# Autodesk Inventor assembly: Stufen Zusammenbau
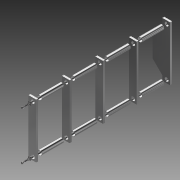
[picture p0: Inventor's stored thumbnail of the model, 180x180]
Saved by Autodesk Inventor 2019 (Build 230136000, 136)
## iProperties
Created: 2020-05-13
Part Number: Stufen Zusammenbau
Material: Generisch
Document SubType Name: Assembly
Designer: seele
Author: seele
## Documents named in this file (7)
- F:\Desktop\Neuer Ordner\Zubehör\Badeleiter\Stufen Zusammenbau.iam
- F:\Desktop\Neuer Ordner\Zubehör\Badeleiter\Tritt.ipt
- F:\Desktop\Neuer Ordner\Zubehör\Badeleiter\Tritt oben.ipt
- F:\Desktop\Neuer Ordner\Zubehör\Badeleiter\Stufenrohr.ipt
- C:\Users\seele\Documents\Inventor\Content Center Files\R2019\de-DE\DIN 931-1\DIN 931-1 - M12 x 50.ipt
- C:\Users\seele\Documents\Inventor\Content Center Files\R2019\de-DE\DIN 128\DIN 128 - A12.ipt
- C:\Users\seele\Documents\Inventor\Content Center Files\R2019\de-DE\DIN 9021\DIN 9021 - 13.ipt
## Components (19 placed, 6 different names)
1. Tritt:1 — Fluchtend:1, Fluchtend:6, Passend:1, Passend:9, Passend:30, Passend:31, Passend:32
2. Tritt:2 — Fluchtend:1, Fluchtend:2, Fluchtend:5, Fluchtend:6, Passend:2, Passend:8, Passend:10, Passend:11
3. Tritt:3 — Fluchtend:2, Fluchtend:3, Fluchtend:4, Fluchtend:5, Passend:3, Passend:7, Passend:12, Passend:13
4. Tritt:4 — Fluchtend:3, Fluchtend:4, Fluchtend:7, Fluchtend:8, Passend:6, Passend:14, Passend:15
5. Tritt oben:1 — Fluchtend:7, Fluchtend:8, Passend:4, Passend:5, Passend:16
6. Stufenrohr:1 — Passend:4, Passend:15, Passend:16, Fluchtend:9
7. Stufenrohr:2 — Passend:5, Fluchtend:9
8. Stufenrohr:3 — Passend:6, Fluchtend:10
9. Stufenrohr:4 — Passend:3, Passend:13, Passend:14, Fluchtend:10
10. Stufenrohr:5 — Passend:2, Passend:11, Passend:12, Fluchtend:11
11. Stufenrohr:6 — Passend:7, Fluchtend:11
12. Stufenrohr:7 — Passend:8, Fluchtend:12
13. Stufenrohr:8 — Passend:1, Passend:9, Passend:10, Fluchtend:12
14. DIN 931-1 - ersetzt durch DIN EN 24014 M12 x 50:3 — Passend:25, Passend:30, Fluchtend:13
15. DIN 128 A12:3
16. DIN 9021 13:1 — Passend:25, Passend:32
17. DIN 931-1 - ersetzt durch DIN EN 24014 M12 x 50:4 — Passend:31, Fluchtend:13
18. DIN 128 A12:4
19. DIN 9021 13:2
## Relationships (40: Mate 27, Flush 13)
- Fluchtend:1 [Flush]: Tritt:1 ↔ Tritt:2
- Fluchtend:2 [Flush]: Tritt:2 ↔ Tritt:3
- Fluchtend:3 [Flush]: Tritt:3 ↔ Tritt:4
- Fluchtend:4 [Flush]: Tritt:3 ↔ Tritt:4
- Fluchtend:5 [Flush]: Tritt:2 ↔ Tritt:3
- Fluchtend:6 [Flush]: Tritt:1 ↔ Tritt:2
- Fluchtend:7 [Flush]: Tritt:4 ↔ Tritt oben:1
- Fluchtend:8 [Flush]: Tritt:4 ↔ Tritt oben:1
- Passend:1 [Mate]: Tritt:1 ↔ Stufenrohr:8
- Passend:2 [Mate]: Tritt:2 ↔ Stufenrohr:5
- Passend:3 [Mate]: Tritt:3 ↔ Stufenrohr:4
- Passend:4 [Mate]: Tritt oben:1 ↔ Stufenrohr:1
- Passend:5 [Mate]: Tritt oben:1 ↔ Stufenrohr:2
- Passend:6 [Mate]: Tritt:4 ↔ Stufenrohr:3
- Passend:7 [Mate]: Tritt:3 ↔ Stufenrohr:6
- Passend:8 [Mate]: Tritt:2 ↔ Stufenrohr:7
- Passend:9 [Mate] (50 mm): Tritt:1 ↔ Stufenrohr:8
- Passend:10 [Mate] (50 mm): Tritt:2 ↔ Stufenrohr:8
- Passend:11 [Mate] (50 mm): Tritt:2 ↔ Stufenrohr:5
- Passend:12 [Mate] (50 mm): Tritt:3 ↔ Stufenrohr:5
- Passend:13 [Mate] (50 mm): Tritt:3 ↔ Stufenrohr:4
- Passend:14 [Mate] (50 mm): Tritt:4 ↔ Stufenrohr:4
- Passend:15 [Mate] (50 mm): Tritt:4 ↔ Stufenrohr:1
- Passend:16 [Mate] (50 mm): Tritt oben:1 ↔ Stufenrohr:1
- Fluchtend:9 [Flush]: Stufenrohr:1 ↔ Stufenrohr:2
- Fluchtend:10 [Flush]: Stufenrohr:3 ↔ Stufenrohr:4
- Fluchtend:11 [Flush]: Stufenrohr:5 ↔ Stufenrohr:6
- Fluchtend:12 [Flush]: Stufenrohr:7 ↔ Stufenrohr:8
- [Mate]: DIN 931-1 - ersetzt durch DIN EN 24014 M12 x 50:3 ↔ DIN 128 A12:3
- [Mate] (60 mm): DIN 931-1 - ersetzt durch DIN EN 24014 M12 x 50:3 ↔ DIN 128 A12:3
- [Mate]: DIN 931-1 - ersetzt durch DIN EN 24014 M12 x 50:3 ↔ DIN 9021 13:1
- Passend:25 [Mate] (75 mm): DIN 931-1 - ersetzt durch DIN EN 24014 M12 x 50:3 ↔ DIN 9021 13:1
- [Mate]: DIN 931-1 - ersetzt durch DIN EN 24014 M12 x 50:4 ↔ DIN 128 A12:4
- [Mate] (60 mm): DIN 931-1 - ersetzt durch DIN EN 24014 M12 x 50:4 ↔ DIN 128 A12:4
- [Mate]: DIN 931-1 - ersetzt durch DIN EN 24014 M12 x 50:4 ↔ DIN 9021 13:2
- [Mate] (75 mm): DIN 931-1 - ersetzt durch DIN EN 24014 M12 x 50:4 ↔ DIN 9021 13:2
- Passend:30 [Mate]: Tritt:1 ↔ DIN 931-1 - ersetzt durch DIN EN 24014 M12 x 50:3
- Passend:31 [Mate]: Tritt:1 ↔ DIN 931-1 - ersetzt durch DIN EN 24014 M12 x 50:4
- Fluchtend:13 [Flush]: DIN 931-1 - ersetzt durch DIN EN 24014 M12 x 50:3 ↔ DIN 931-1 - ersetzt durch DIN EN 24014 M12 x 50:4
- Passend:32 [Mate] (30 mm): Tritt:1 ↔ DIN 9021 13:1
## Named parameters: d37_d53 = 0 mm, d38_d54 = 60 mm, d39_d57 = 0 mm, d40_d36 = 75 mm
